# Autodesk Inventor assembly: axis4
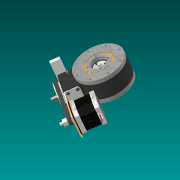
[picture p0: Inventor's stored thumbnail of the model, 180x180]
Saved by Autodesk Inventor 2020 (Build 240168000, 168)
## iProperties
Created: 2020-05-24
Part Number: axis4
Document SubType Name: Assembly
Designer: Svend
Author: Svend
## Documents named in this file (20)
- D:\github_gedeeld\BeerMinder\3D-model\axis4\axis4.iam
- D:\github_gedeeld\BeerMinder\3D-model\pulleys\GT2 Timing Pulley 60T - 8mm as.ipt
- D:\github_gedeeld\BeerMinder\3D-model\stepper motors\42BYG Stepper Motor.ipt
- D:\github_gedeeld\BeerMinder\3D-model\pulleys\GT2 Pulley 16T - 5mm as.ipt
- D:\github_gedeeld\BeerMinder\3D-model\pulleys\Tandriem16naar60T.ipt
- D:\github_gedeeld\BeerMinder\3D-model\Base (Axis 1)\asArm2.ipt
- D:\github_gedeeld\BeerMinder\3D-model\axis4\steppermount.ipt
- D:\github_gedeeld\BeerMinder\3D-model\axis4\stepperspacer.ipt
- D:\github_gedeeld\BeerMinder\3D-model\boutjesEnMoertjes\ISO 7380-1 - M3 x 10.ipt
- D:\github_gedeeld\BeerMinder\3D-model\boutjesEnMoertjes\ISO 4035 - M3 - ISO.ipt
- D:\github_gedeeld\BeerMinder\3D-model\boutjesEnMoertjes\ISO 7380-1 - M3 x 8.ipt
- D:\github_gedeeld\BeerMinder\3D-model\bearings\conische lager.ipt
- D:\github_gedeeld\BeerMinder\3D-model\bearings\insertLager.ipt
- D:\github_gedeeld\BeerMinder\3D-model\boutjesEnMoertjes\ISO 4762 - M4 x 40ISO.ipt
- D:\github_gedeeld\BeerMinder\3D-model\Base (Axis 1)\as4mount v2.ipt
- D:\github_gedeeld\BeerMinder\3D-model\axis4\asmountAs4klein.ipt
- D:\github_gedeeld\BeerMinder\3D-model\axis4\spacerHex.ipt
- D:\github_gedeeld\BeerMinder\3D-model\bearings\slew bearing 80v2\Slew Bearing 80v2.iam
- D:\github_gedeeld\BeerMinder\3D-model\boutjesEnMoertjes\ISO 10642 - M3x20.ipt
- C:\Users\stefa\Documents\Inventor\Content Center Files\R2020\en-US\ISO 7380-1\ISO 7380-1 - M3 x 25.ipt
## Components (57 placed, 19 different names)
1. as4mount v2:1 — Mate:9, Angle:2, Flush:8, Mate:17, Mate:18, Mate:31, Mate:32, Mate:33, Mate:34, Mate:35, Mate:36, Mate:37, Mate:39, Mate:43, Mate:38, Flush:55, Mate:52, Mate:53, Mate:54, Mate:55, Mate:56, Mate:58, Mate:59, Mate:60, Mate:61, Mate:62, Mate:63, Mate:64, Mate:65, Flush:57, Mate:68, Mate:70, Mate:71, Mate:80, Angle:4, Flush:61, Flush:62, Mate:81, Mate:82, Mate:83, Mate:84, Mate:85, Mate:86
2. GT2 Timing Pulley 60T - 8mm as:1 — Mate:7, Mate:8, Mate:43, Mate:50, Angle:3
3. 42BYG Stepper Motor:1 — Mate:13, Angle:2, Flush:8, Mate:19, Mate:20, Mate:21, Mate:23, Mate:24, Mate:25, Mate:26
4. GT2 Pulley 16T - 5mm as:1 — Mate:11, Mate:12, Mate:13
5. Tandriem16naar60T:1 — Mate:7, Mate:8, Mate:11, Mate:12
6. asArm2:1 — Mate:49, Mate:50, Mate:51
7. asmountAs4klein:1 — Mate:9, Mate:80, Angle:4, Flush:61, Flush:62
8. steppermount:1 — Mate:17, Mate:18, Mate:27, Mate:28, Mate:29, Mate:30, Insert:1, Insert:2, Insert:3, Insert:4, Mate:44, Angle:3
9. stepperspacer:1 — Mate:19, Mate:20, Mate:21, Mate:44
10. conische lager:1 — Mate:39, Mate:49, Mate:51, Flush:56
11. insertLager:1 — Flush:55, Mate:52, Mate:53, Flush:56
12. ISO 4762 M4 x 40:1 — Mate:54, Mate:55
13. Slew Bearing 80v2:1 [sub-assembly] — Mate:56, Mate:66, Mate:71, Mate:72, Mate:73, Mate:74, Mate:75, Insert:13, Insert:14, Insert:15, Insert:16, Insert:17, Insert:18, Insert:19, Insert:20
14. spacerHex:1 — Mate:62, Mate:63, Flush:60
15. spacerHex:2 — Mate:64, Mate:65, Flush:57, Flush:58, Flush:60, Mate:66, Mate:69
16. spacerHex:3 — Mate:60, Mate:61, Flush:59
17. spacerHex:4 — Mate:58, Mate:59, Flush:58, Flush:59
18. Slew Bearing 80v2:2 [sub-assembly] — Mate:68, Mate:69, Mate:70, Mate:76, Mate:77, Mate:78, Mate:79, Insert:5, Insert:6, Insert:7, Insert:8, Insert:9, Insert:10, Insert:11, Insert:12
19. ISO 4035 M3:20 — Insert:20
20. ISO 4035 M3:19 — Insert:19
21. ISO 4035 M3:18 — Insert:18
22. ISO 4035 M3:17 — Insert:17
23. ISO 4035 M3:16 — Insert:16
24. ISO 4035 M3:15 — Insert:15
25. ISO 4035 M3:14 — Insert:14
26. ISO 4035 M3:13 — Insert:13
27. ISO 4035 M3:12 — Insert:12
28. ISO 4035 M3:11 — Insert:11
29. ISO 4035 M3:10 — Insert:10
30. ISO 4035 M3:9 — Insert:9
31. ISO 4035 M3:8 — Insert:8
32. ISO 4035 M3:7 — Insert:7
33. ISO 4035 M3:6 — Insert:6
34. ISO 4035 M3:5 — Insert:5
35. ISO 7380-1 M3 x 25:3 — Mate:85, Mate:86
36. ISO 7380-1 M3 x 25:2 — Mate:83, Mate:84
37. ISO 7380-1 M3 x 25:1 — Mate:81, Mate:82
38. ISO 10642 M3x20:8 — Mate:79
39. ISO 10642 M3x20:7 — Mate:78
40. ISO 10642 M3x20:6 — Mate:77
41. ISO 10642 M3x20:5 — Mate:76
42. ISO 10642 M3x20:4 — Mate:75
43. ISO 10642 M3x20:3 — Mate:74
44. ISO 10642 M3x20:2 — Mate:73
45. ISO 10642 M3x20:1 — Mate:72
46. ISO 7380-1 M3 x 10:1 — Mate:23, Mate:29
47. ISO 7380-1 M3 x 10:2 — Mate:26, Mate:27
48. ISO 7380-1 M3 x 10:3 — Mate:24, Mate:30
49. ISO 7380-1 M3 x 10:4 — Mate:25, Mate:28
50. ISO 4035 M3:1 — Mate:34, Mate:37
51. ISO 4035 M3:2 — Mate:35, Mate:36
52. ISO 4035 M3:3 — Mate:33, Mate:38
53. ISO 4035 M3:4 — Mate:31, Mate:32
54. ISO 7380-1 M3 x 8:1 — Insert:1
55. ISO 7380-1 M3 x 8:2 — Insert:2
56. ISO 7380-1 M3 x 8:3 — Insert:3
57. ISO 7380-1 M3 x 8:4 — Insert:4
## Relationships (98: Mate 66, Insert 20, Flush 9, Angle 3)
- Mate:7: GT2 Timing Pulley 60T - 8mm as:1 ↔ Tandriem16naar60T:1
- Mate:8 (0.5 mm): GT2 Timing Pulley 60T - 8mm as:1 ↔ Tandriem16naar60T:1
- Mate:9: as4mount v2:1 ↔ asmountAs4klein:1
- Mate:11: GT2 Pulley 16T - 5mm as:1 ↔ Tandriem16naar60T:1
- Mate:12 (0.5 mm): GT2 Pulley 16T - 5mm as:1 ↔ Tandriem16naar60T:1
- Mate:13: 42BYG Stepper Motor:1 ↔ GT2 Pulley 16T - 5mm as:1
- Angle:2 (180 deg): as4mount v2:1 ↔ 42BYG Stepper Motor:1
- Flush:8: as4mount v2:1 ↔ 42BYG Stepper Motor:1
- Mate:17: as4mount v2:1 ↔ steppermount:1
- Mate:18: as4mount v2:1 ↔ steppermount:1
- Mate:19: 42BYG Stepper Motor:1 ↔ stepperspacer:1
- Mate:20: 42BYG Stepper Motor:1 ↔ stepperspacer:1
- Mate:21: 42BYG Stepper Motor:1 ↔ stepperspacer:1
- Mate:23: 42BYG Stepper Motor:1 ↔ ISO 7380-1 M3 x 10:1
- Mate:24: 42BYG Stepper Motor:1 ↔ ISO 7380-1 M3 x 10:3
- Mate:25: 42BYG Stepper Motor:1 ↔ ISO 7380-1 M3 x 10:4
- Mate:26: 42BYG Stepper Motor:1 ↔ ISO 7380-1 M3 x 10:2
- Mate:27: steppermount:1 ↔ ISO 7380-1 M3 x 10:2
- Mate:28: steppermount:1 ↔ ISO 7380-1 M3 x 10:4
- Mate:29: steppermount:1 ↔ ISO 7380-1 M3 x 10:1
- Mate:30: steppermount:1 ↔ ISO 7380-1 M3 x 10:3
- Mate:31: as4mount v2:1 ↔ ISO 4035 M3:4
- Mate:32: as4mount v2:1 ↔ ISO 4035 M3:4
- Mate:33: as4mount v2:1 ↔ ISO 4035 M3:3
- Mate:34: as4mount v2:1 ↔ ISO 4035 M3:1
- Mate:35: as4mount v2:1 ↔ ISO 4035 M3:2
- Mate:36: as4mount v2:1 ↔ ISO 4035 M3:2
- Mate:37: as4mount v2:1 ↔ ISO 4035 M3:1
- Mate:38: as4mount v2:1 ↔ ISO 4035 M3:3
- Insert:1: steppermount:1 ↔ ISO 7380-1 M3 x 8:1
- Insert:2: steppermount:1 ↔ ISO 7380-1 M3 x 8:2
- Insert:3: steppermount:1 ↔ ISO 7380-1 M3 x 8:3
- Insert:4: steppermount:1 ↔ ISO 7380-1 M3 x 8:4
- Mate:39: as4mount v2:1 ↔ conische lager:1
- Mate:43: as4mount v2:1 ↔ GT2 Timing Pulley 60T - 8mm as:1
- Mate:44: steppermount:1 ↔ stepperspacer:1
- Mate:49: asArm2:1 ↔ conische lager:1
- Mate:50: GT2 Timing Pulley 60T - 8mm as:1 ↔ asArm2:1
- Angle:3 (0 deg): GT2 Timing Pulley 60T - 8mm as:1 ↔ steppermount:1
- Mate:51 (-11 mm): asArm2:1 ↔ conische lager:1
- Flush:55: as4mount v2:1 ↔ insertLager:1
- Mate:52 (0.05 mm): as4mount v2:1 ↔ insertLager:1
- Mate:53 (0.05 mm): as4mount v2:1 ↔ insertLager:1
- Mate:54: as4mount v2:1 ↔ ISO 4762 M4 x 40:1
- Mate:55: as4mount v2:1 ↔ ISO 4762 M4 x 40:1
- Flush:56: conische lager:1 ↔ insertLager:1
- Mate:56: as4mount v2:1 ↔ Slew Bearing 80v2:1
- Mate:58: as4mount v2:1 ↔ spacerHex:4
- Mate:59: as4mount v2:1 ↔ spacerHex:4
- Mate:60: as4mount v2:1 ↔ spacerHex:3
- Mate:61: as4mount v2:1 ↔ spacerHex:3
- Mate:62: as4mount v2:1 ↔ spacerHex:1
- Mate:63: as4mount v2:1 ↔ spacerHex:1
- Mate:64: as4mount v2:1 ↔ spacerHex:2
- Mate:65: as4mount v2:1 ↔ spacerHex:2
- Flush:57 (8.1995 mm): as4mount v2:1 ↔ spacerHex:2
- Flush:58: spacerHex:2 ↔ spacerHex:4
- Flush:59: spacerHex:3 ↔ spacerHex:4
- Flush:60: spacerHex:1 ↔ spacerHex:2
- Mate:66: Slew Bearing 80v2:1 ↔ spacerHex:2
- Mate:68: as4mount v2:1 ↔ Slew Bearing 80v2:2
- Mate:69: spacerHex:2 ↔ Slew Bearing 80v2:2
- Mate:70: as4mount v2:1 ↔ Slew Bearing 80v2:2
- Mate:71: as4mount v2:1 ↔ Slew Bearing 80v2:1
- Mate:72: Slew Bearing 80v2:1 ↔ ISO 10642 M3x20:1
- Mate:73: Slew Bearing 80v2:1 ↔ ISO 10642 M3x20:2
- Mate:74: Slew Bearing 80v2:1 ↔ ISO 10642 M3x20:3
- Mate:75: Slew Bearing 80v2:1 ↔ ISO 10642 M3x20:4
- Mate:76: Slew Bearing 80v2:2 ↔ ISO 10642 M3x20:5
- Mate:77: Slew Bearing 80v2:2 ↔ ISO 10642 M3x20:6
- Mate:78: Slew Bearing 80v2:2 ↔ ISO 10642 M3x20:7
- Mate:79: Slew Bearing 80v2:2 ↔ ISO 10642 M3x20:8
- Mate:80: as4mount v2:1 ↔ asmountAs4klein:1
- Angle:4 (240 deg): as4mount v2:1 ↔ asmountAs4klein:1
- Flush:61: as4mount v2:1 ↔ asmountAs4klein:1
- Flush:62: as4mount v2:1 ↔ asmountAs4klein:1
- Mate:81: as4mount v2:1 ↔ ISO 7380-1 M3 x 25:1
- Mate:82: as4mount v2:1 ↔ ISO 7380-1 M3 x 25:1
- Mate:83: as4mount v2:1 ↔ ISO 7380-1 M3 x 25:2
- Mate:84: as4mount v2:1 ↔ ISO 7380-1 M3 x 25:2
- Mate:85: as4mount v2:1 ↔ ISO 7380-1 M3 x 25:3
- Mate:86: as4mount v2:1 ↔ ISO 7380-1 M3 x 25:3
- Insert:5: Slew Bearing 80v2:2 ↔ ISO 4035 M3:5
- Insert:6: Slew Bearing 80v2:2 ↔ ISO 4035 M3:6
- Insert:7: Slew Bearing 80v2:2 ↔ ISO 4035 M3:7
- Insert:8: Slew Bearing 80v2:2 ↔ ISO 4035 M3:8
- Insert:9: Slew Bearing 80v2:2 ↔ ISO 4035 M3:9
- Insert:10: Slew Bearing 80v2:2 ↔ ISO 4035 M3:10
- Insert:11: Slew Bearing 80v2:2 ↔ ISO 4035 M3:11
- Insert:12: Slew Bearing 80v2:2 ↔ ISO 4035 M3:12
- Insert:13: Slew Bearing 80v2:1 ↔ ISO 4035 M3:13
- Insert:14: Slew Bearing 80v2:1 ↔ ISO 4035 M3:14
- Insert:15: Slew Bearing 80v2:1 ↔ ISO 4035 M3:15
- Insert:16: Slew Bearing 80v2:1 ↔ ISO 4035 M3:16
- Insert:17: Slew Bearing 80v2:1 ↔ ISO 4035 M3:17
- Insert:18: Slew Bearing 80v2:1 ↔ ISO 4035 M3:18
- Insert:19: Slew Bearing 80v2:1 ↔ ISO 4035 M3:19
- Insert:20: Slew Bearing 80v2:1 ↔ ISO 4035 M3:20
